# Autodesk Inventor assembly: stand3.0
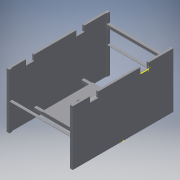
[picture p0: Inventor's stored thumbnail of the model, 180x180]
Saved by Autodesk Inventor 2019 (Build 230136000, 136)
## iProperties
Created: 2020-02-18
Part Number: stand3.0
Document SubType Name: Assembly
Designer: admin
Author: admin
## Documents named in this file (4)
- C:\Users\admin\Desktop\Exploration\stand3.0.iam
- C:\Users\admin\Desktop\Exploration\stand2.0.ipt
- C:\Users\admin\Desktop\Exploration\030 motor mount-2-Production.ipt
- C:\Users\admin\Desktop\Exploration\DC assembly.iam
## Components (3 placed, 3 different names)
1. stand2.0:1 — Rigid:1, Rigid:3
2. 030 motor mount-2-Production:1 — Tangent:1, Tangent:2, Mate:1, Cylindrical:1, Rigid:1, Mate:2, Rigid:2, Rigid:3
3. DC assembly:1 [sub-assembly] — Tangent:1, Tangent:2, Mate:1, Cylindrical:1, Mate:2, Rigid:2
## Relationships (8: WeldJoint 3, Tangent 2, Mate 2, CylindricalJoint 1)
- Tangent:1: 030 motor mount-2-Production:1 ↔ DC assembly:1
- Tangent:2: 030 motor mount-2-Production:1 ↔ DC assembly:1
- Mate:1: 030 motor mount-2-Production:1 ↔ DC assembly:1
- Cylindrical:1: 030 motor mount-2-Production:1 ↔ DC assembly:1
- Rigid:1 [WeldJoint]: stand2.0:1 ↔ 030 motor mount-2-Production:1
- Mate:2: 030 motor mount-2-Production:1 ↔ DC assembly:1
- Rigid:2 [WeldJoint]: 030 motor mount-2-Production:1 ↔ DC assembly:1
- Rigid:3 [WeldJoint]: stand2.0:1 ↔ 030 motor mount-2-Production:1
